# Autodesk Inventor assembly: Wasserverteiler
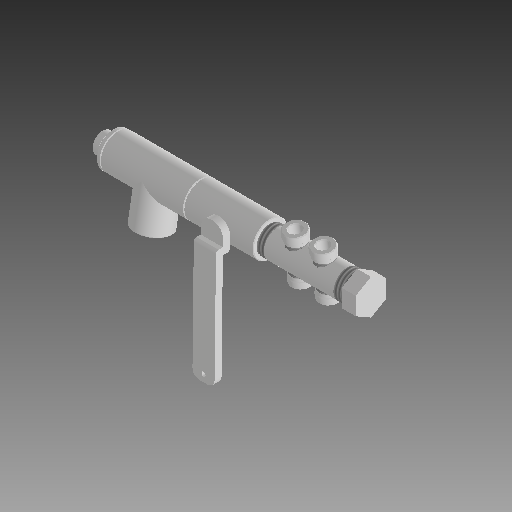
[picture p0: Inventor's stored thumbnail of the model, 512x512]
Saved by Autodesk Inventor 2021 (Build 250183000, 183)
## iProperties
Created: 2022-02-28
Part Number: Wasserverteiler
Document SubType Name: Assembly
Designer: lukas
Stock Number: Wasserventil
Author: lukas
## Documents named in this file (8)
- C:\Users\lukas\OneDrive - HTBLA Kaindorf\Diplomarbeit\Mechanik\InventorKonstruktion\Wasserverteiler.iam
- C:\Users\lukas\OneDrive - HTBLA Kaindorf\Diplomarbeit\Mechanik\InventorKonstruktion\VerteilerVerschluss.ipt
- C:\Users\lukas\OneDrive - HTBLA Kaindorf\Diplomarbeit\Mechanik\InventorKonstruktion\Wasserverteiler1.ipt
- C:\Users\lukas\OneDrive - HTBLA Kaindorf\Diplomarbeit\Mechanik\InventorKonstruktion\Wasserverteiler2.ipt
- C:\Users\lukas\OneDrive - HTBLA Kaindorf\Diplomarbeit\Mechanik\InventorKonstruktion\Verbindungsstück.ipt
- C:\Users\lukas\OneDrive - HTBLA Kaindorf\Diplomarbeit\Mechanik\InventorKonstruktion\Schlauchsteckverbindung.ipt
- C:\Users\lukas\OneDrive - HTBLA Kaindorf\Diplomarbeit\Mechanik\InventorKonstruktion\VentilNukleator2.ipt
- C:\Users\lukas\OneDrive - HTBLA Kaindorf\Diplomarbeit\Mechanik\InventorKonstruktion\VentilNukleator.ipt
## Components (11 placed, 7 different names)
1. Wasserverteiler1:1 — Zylindrisch:1, Passend:1, Starr:1, Starr:2, Starr:3, Starr:4, Drehbar:4
2. Wasserverteiler2:1 — Zylindrisch:1, Passend:1
3. Schlauchsteckverbindung:1 — Starr:1
4. Schlauchsteckverbindung:2 — Starr:2
5. Schlauchsteckverbindung:3 — Starr:3
6. Schlauchsteckverbindung:4 — Starr:4
7. VerteilerVerschluss:1 — Drehbar:1, Drehbar:2
8. Schlauchsteckverbindung:5 — Drehbar:2
9. Verbindungsstück:1 — Drehbar:1, Drehbar:3
10. VentilNukleator2:1 — Starr:5
11. VentilNukleator:1 — Drehbar:3, Drehbar:4, Starr:5
## Relationships (11: WeldJoint 5, RevoluteJoint 4, CylindricalJoint 1, Mate 1)
- Zylindrisch:1 [CylindricalJoint]: Wasserverteiler1:1 ↔ Wasserverteiler2:1
- Passend:1 [Mate] (-2 mm): Wasserverteiler1:1 ↔ Wasserverteiler2:1
- Starr:1 [WeldJoint] (-7 mm): Wasserverteiler1:1 ↔ Schlauchsteckverbindung:1
- Starr:2 [WeldJoint] (-7 mm): Wasserverteiler1:1 ↔ Schlauchsteckverbindung:2
- Starr:3 [WeldJoint] (-7 mm): Wasserverteiler1:1 ↔ Schlauchsteckverbindung:3
- Starr:4 [WeldJoint] (-7 mm): Wasserverteiler1:1 ↔ Schlauchsteckverbindung:4
- Drehbar:1 [RevoluteJoint] (-5 mm): VerteilerVerschluss:1 ↔ Verbindungsstück:1
- Drehbar:2 [RevoluteJoint] (7 mm): VerteilerVerschluss:1 ↔ Schlauchsteckverbindung:5
- Drehbar:3 [RevoluteJoint] (-10 mm): Verbindungsstück:1 ↔ VentilNukleator:1
- Drehbar:4 [RevoluteJoint] (10 mm): Wasserverteiler1:1 ↔ VentilNukleator:1
- Starr:5 [WeldJoint]: VentilNukleator2:1 ↔ VentilNukleator:1
